# Autodesk Inventor assembly: ABD_Slider_Set
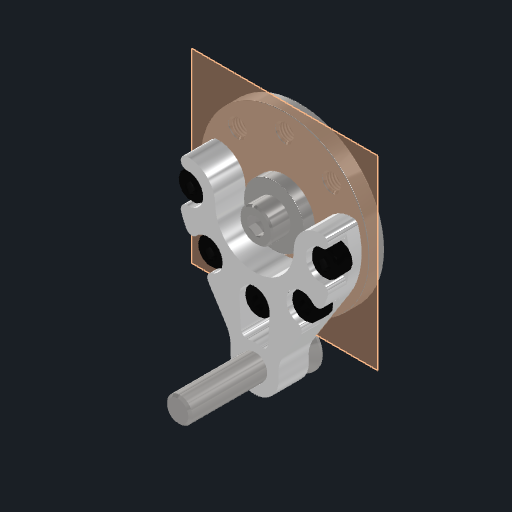
[picture p0: Inventor's stored thumbnail of the model, 512x512]
Saved by Autodesk Inventor 2024.3 (Build 283343000, 343)
## iProperties
Created: 2024-02-15
Part Number: ABD_Slider_Set
Document SubType Name: Assembly
Designer: ASUS
Author: ASUS
## Documents named in this file (6)
- C:\Users\ASUS\Desktop\Anti_Backlash_Structure_OP\v2_Frame\ABD_Slider_Set_v2.iam
- C:\Users\ASUS\Desktop\2024_Robit_Hardware\ROBOCUP_2024_eindhoven\부품\ROBOTIS(Inventor 2023 ver.)\혼\64-106Horn.ipt
- C:\Users\ASUS\Desktop\Anti_Backlash_Structure_OP\v2_Frame\Slider_crank_horn_v2.ipt
- C:\Users\ASUS\Desktop\ABD_2024_Eindhoven\MISUMI\CSH-STN-M3-10_203.ipt
- C:\Users\ASUS\Desktop\ABD_2024_Eindhoven\MISUMI\CSHCS-SUSTBS-M4-20_214.ipt
- C:\Users\ASUS\Desktop\ABD_2024_Eindhoven\MISUMI\4mm_ABD_set.iam
## Components (5 placed, 5 different names)
1. 64-106Horn:1 — 삽입:3, 삽입:6, 메이트:1
2. Slider_crank_horn_v2:1 — 삽입:5, 삽입:6, 메이트:1, 삽입:7, 메이트:2
3. CSH-STN-M3-10_203:1 — 삽입:3
4. CSHCS-SUSTBS-M4-20_214:1 — 삽입:5
5. 4mm_ABD_set:1 [sub-assembly] — 삽입:7, 메이트:2
## Relationships (6: Insert 4, Mate 2)
- 삽입:3 [Insert]: 64-106Horn:1 ↔ CSH-STN-M3-10_203:1
- 삽입:5 [Insert]: Slider_crank_horn_v2:1 ↔ CSHCS-SUSTBS-M4-20_214:1
- 삽입:6 [Insert]: 64-106Horn:1 ↔ Slider_crank_horn_v2:1
- 메이트:1 [Mate]: 64-106Horn:1 ↔ Slider_crank_horn_v2:1
- 삽입:7 [Insert]: Slider_crank_horn_v2:1 ↔ 4mm_ABD_set:1
- 메이트:2 [Mate]: Slider_crank_horn_v2:1 ↔ 4mm_ABD_set:1
